# Autodesk Inventor assembly: A2017_T5_03
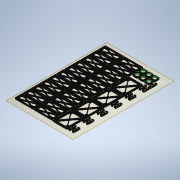
[picture p0: Inventor's stored thumbnail of the model, 180x180]
Saved by Autodesk Inventor 2022 (Build 260153000, 153)
## iProperties
Created: 2022-09-28
Part Number: A2017_T5_03
Document SubType Name: Assembly
Designer: Masato
Author: Masato
## Documents named in this file (6)
- C:\Users\ヨコオリク\Documents\CITBrains\SUSTAINA-OP\Cam\A2017_T5\A2017_T5_03.iam
- C:\Users\ヨコオリク\Documents\CITBrains\SUSTAINA-OP\Cam\DisposableBoard.ipt
- C:\Users\ヨコオリク\Documents\CITBrains\SUSTAINA-OP\LowerBody\Link\FrontLink_diagonal.ipt
- C:\Users\ヨコオリク\Documents\CITBrains\SUSTAINA-OP\LowerBody\Link\BackLink_diagonal.ipt
- C:\Users\ヨコオリク\Documents\CITBrains\SUSTAINA-OP\LowerBody\Knee\Knee_clamp.ipt
- C:\Users\ヨコオリク\Documents\CITBrains\SUSTAINA-OP\LowerBody\Foot\Foot_root_block.ipt
## Components (46 placed, 5 different names)
1. DisposableBoard:1 — フラッシュ:1, フラッシュ:2, フラッシュ:3, フラッシュ:4, フラッシュ:5, フラッシュ:6, フラッシュ:7, フラッシュ:8, 正接:1, 正接:2
2. Foot_root_block:23 — メイト:5, 正接:4, メイト:6
3. BackLink_diagonal:1 — フラッシュ:5, フラッシュ:6
4. BackLink_diagonal:2 — メイト:2
5. BackLink_diagonal:3
6. BackLink_diagonal:4
7. BackLink_diagonal:5
8. BackLink_diagonal:6
9. BackLink_diagonal:7
10. BackLink_diagonal:8
11. BackLink_diagonal:9
12. BackLink_diagonal:10
13. BackLink_diagonal:11
14. BackLink_diagonal:12
15. BackLink_diagonal:13
16. BackLink_diagonal:14
17. BackLink_diagonal:15
18. BackLink_diagonal:16
19. BackLink_diagonal:17
20. BackLink_diagonal:18
21. BackLink_diagonal:19
22. BackLink_diagonal:20
23. BackLink_diagonal:21
24. BackLink_diagonal:22 — 正接:3
25. FrontLink_diagonal:1 — メイト:1, フラッシュ:8, メイト:2, メイト:3
26. FrontLink_diagonal:2
27. FrontLink_diagonal:3
28. FrontLink_diagonal:4
29. Foot_root_block:1 — フラッシュ:7, メイト:3
30. Foot_root_block:2
31. Foot_root_block:5
32. Foot_root_block:6
33. Foot_root_block:9
34. Foot_root_block:10
35. Foot_root_block:13
36. Foot_root_block:14
37. Foot_root_block:17
38. Foot_root_block:18
39. Foot_root_block:21
40. Foot_root_block:22 — メイト:6
41. Knee_clamp:1 — メイト:4, 正接:1, 正接:2, 正接:3
42. Knee_clamp:2
43. Knee_clamp:3
44. Knee_clamp:4
45. Knee_clamp:5
46. Knee_clamp:6 — 正接:4
## Component patterns: (22 elements, first: BackLink_diagonal:1), (4 elements, first: FrontLink_diagonal:1), (22 elements, first: Foot_root_block:1), (6 elements, first: Knee_clamp:1)
## Relationships (18: Flush 8, Mate 6, Tangent 4)
- フラッシュ:1 [Flush]: DisposableBoard:1
- フラッシュ:2 [Flush]: DisposableBoard:1
- フラッシュ:3 [Flush]: DisposableBoard:1
- フラッシュ:4 [Flush]: DisposableBoard:1
- フラッシュ:5 [Flush] (2 mm): DisposableBoard:1 ↔ BackLink_diagonal:1
- フラッシュ:6 [Flush] (2 mm): DisposableBoard:1 ↔ BackLink_diagonal:1
- フラッシュ:7 [Flush] (2 mm): DisposableBoard:1 ↔ Foot_root_block:1
- メイト:1 [Mate]: FrontLink_diagonal:1
- フラッシュ:8 [Flush] (-2 mm): DisposableBoard:1 ↔ FrontLink_diagonal:1
- メイト:2 [Mate] (2.1 mm): BackLink_diagonal:2 ↔ FrontLink_diagonal:1
- メイト:3 [Mate] (2.1 mm): FrontLink_diagonal:1 ↔ Foot_root_block:1
- メイト:4 [Mate]: Knee_clamp:1
- 正接:1 [Tangent] (3 mm): DisposableBoard:1 ↔ Knee_clamp:1
- 正接:2 [Tangent] (3 mm): DisposableBoard:1 ↔ Knee_clamp:1
- 正接:3 [Tangent] (2.1 mm): BackLink_diagonal:22 ↔ Knee_clamp:1
- メイト:5 [Mate]: Foot_root_block:23
- 正接:4 [Tangent] (2.5 mm): Foot_root_block:23 ↔ Knee_clamp:6
- メイト:6 [Mate] (2.1 mm): Foot_root_block:23 ↔ Foot_root_block:22
